# Autodesk Inventor assembly: structure
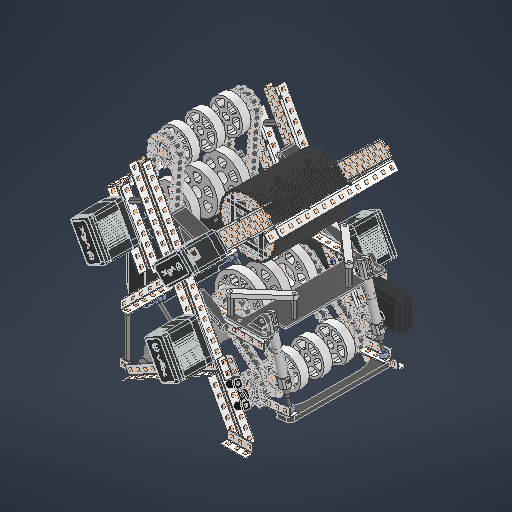
[picture p0: Inventor's stored thumbnail of the model, 512x512]
Saved by Autodesk Inventor 2025.2 (Build 292293000, 293)
## iProperties
Created: 2025-12-03
Part Number: structure
Document SubType Name: Assembly
Designer: cloudy
Mass: 4703.07 g
Surface Area: 21659.1 cm^2
Volume: 2960.96 cm^3
Density: 1.58836 g/cm^3
Author: cloudy
## Documents named in this file (47)
- C:\Users\cloudy\Documents\GitHub\aura-cad\15\structure.iam
- C:\Users\cloudy\Documents\GitHub\aura-cad\!lib\Structure\C Channel\Aluminum 1x3x1 Half\Alu C Half 1x3x1x3.ipt
- C:\Users\cloudy\Documents\GitHub\aura-cad\!lib\Structure\C Channel\Aluminum 1x2x1\Alu C 1x2x1x26.ipt
- C:\Users\cloudy\Documents\GitHub\aura-cad\!lib\Structure\C Channel\Aluminum 1x3x1 Half\Alu C Half 1x3x1x2.ipt
- C:\Users\cloudy\Documents\GitHub\aura-cad\!lib\Structure\C Channel\Aluminum 1x3x1 Half\Alu C Half 1x3x1x12.ipt
- C:\Users\cloudy\Documents\GitHub\aura-cad\!lib\Electronics\Motors with Screws.iam
- C:\Users\cloudy\Documents\GitHub\aura-cad\!lib\Electronics\Motors with Screws\AluM-StarS.iam
- C:\Users\cloudy\Documents\GitHub\aura-cad\!lib\Structure\C Channel\Aluminum 1x2x1\Alu C 1x2x1x14.ipt
- C:\Users\cloudy\Documents\GitHub\aura-cad\15\angleblock.ipt
- C:\Users\cloudy\Documents\GitHub\aura-cad\!lib\Motion\Shaft LS\LS Pillow Bearing Block.ipt
- C:\Users\cloudy\Documents\GitHub\aura-cad\!lib\Structure\C Channel\Aluminum 1x3x1 Half\Alu C Half 1x3x1x17.ipt
- C:\Users\cloudy\Documents\GitHub\aura-cad\!lib\Structure\Standoff\Standoff 1.00.ipt
- C:\Users\cloudy\Documents\GitHub\aura-cad\!lib\Structure\Standoff.ipt
- C:\Users\cloudy\Documents\GitHub\aura-cad\!lib\Structure\C Channel\Aluminum 1x3x1 Half\Alu C Half 1x3x1x8.ipt
- C:\Users\cloudy\Documents\GitHub\aura-cad\15\middlebrace.ipt
- C:\Users\cloudy\Documents\GitHub\aura-cad\15\angleblock_MIR.ipt
- C:\Users\cloudy\Documents\GitHub\aura-cad\15\middlebrace_MIR.ipt
- C:\Users\cloudy\Documents\GitHub\aura-cad\15\ramp.ipt
- C:\Users\cloudy\Documents\GitHub\aura-cad\!lib\Structure\C Channel\Aluminum 1x2x1\Alu C 1x2x1x8.ipt
- C:\Users\cloudy\Documents\GitHub\aura-cad\!lib\Motion\Spacers\Spacer Nylon .375 OD\NSpacer .375 OD x .500.ipt
- C:\Users\cloudy\Documents\GitHub\aura-cad\!lib\Motion\Spacers\Spacer Nylon .375 OD.ipt
- C:\Users\cloudy\Documents\GitHub\aura-cad\!lib\Motion\Spacers\Spacer Nylon .375 OD\NSpacer .375 OD x .125.ipt
- C:\Users\cloudy\Documents\GitHub\aura-cad\!lib\Electronics\V5 Simple Brain.ipt
- C:\Users\cloudy\Documents\GitHub\aura-cad\!lib\Motion\Pneumatics\Legacy - SMC Pneumatics\Reservoir.ipt
- C:\Users\cloudy\Documents\GitHub\aura-cad\!lib\Electronics\V5 Simple Battery.ipt
- C:\Users\cloudy\Documents\GitHub\aura-cad\15\3.157 roller.iam
- C:\Users\cloudy\Documents\GitHub\aura-cad\15\midroller.iam
- C:\Users\cloudy\Documents\GitHub\aura-cad\!lib\Motion\Shaft LS\Shaft Collar Metal\Shaft Collar No Screw.iam
- C:\Users\cloudy\Documents\GitHub\aura-cad\!lib\Motion\Shaft LS\Shaft Collar Metal.iam
- C:\Users\cloudy\Documents\GitHub\aura-cad\15\30 stroke 10 bore\CJ2D10-30Z(0_0).iam
- C:\Users\cloudy\Documents\GitHub\aura-cad\!lib\Structure\Hardware\Nut Keps.ipt
- C:\Users\cloudy\Documents\GitHub\aura-cad\!lib\Motion\Spacers\Spacer Nylon .375 OD\NSpacer .375 OD x .375.ipt
- C:\Users\cloudy\Documents\GitHub\aura-cad\!lib\Motion\Spacers\Washer Steel\SWasher .375 OD x .031250.ipt
- C:\Users\cloudy\Documents\GitHub\aura-cad\!lib\Motion\Spacers\Washer Steel.ipt
- C:\Users\cloudy\Documents\GitHub\aura-cad\!lib\Motion\Shaft LS\Bearing Flat.ipt
- C:\Users\cloudy\Documents\GitHub\aura-cad\!lib\Structure\Hardware\Nut Nylock.ipt
- C:\Users\cloudy\Documents\GitHub\aura-cad\15\back lower roller.iam
- C:\Users\cloudy\Documents\GitHub\aura-cad\15\intake second stage.iam
- C:\Users\cloudy\Documents\GitHub\aura-cad\15\top roller.iam
- C:\Users\cloudy\Documents\GitHub\aura-cad\15\chain 3.256.iam
- C:\Users\cloudy\Documents\GitHub\aura-cad\15\chain 3.48.iam
- C:\Users\cloudy\Documents\GitHub\aura-cad\15\thingy.ipt
- C:\Users\cloudy\Documents\GitHub\aura-cad\!lib\Structure\Standoff\Standoff 2.00.ipt
- C:\Users\cloudy\Documents\GitHub\aura-cad\!lib\Structure\Standoff\Standoff 2.50.ipt
- C:\Users\cloudy\Documents\GitHub\aura-cad\!lib\Structure\C Channel\Aluminum 1x3x1 Half\Alu C Half 1x3x1x6.ipt
- C:\Users\cloudy\Documents\GitHub\aura-cad\15\parkbar.ipt
- C:\Users\cloudy\Documents\GitHub\aura-cad\!lib\Miscellaneous\iw_metal_02.bmp
## Components (91 placed, 40 different names)
1. Alu C Half 1x3x1x3:1 — Insert:2
2. Alu C 1x2x1x26:1 — Insert:2, Insert:4, Insert:6, Mate:3, Insert:7, Mate:4, Insert:9, Insert:11, Mate:5, Insert:12, Mate:6, Insert:15, Insert:18, Insert:19, Insert:43, Insert:49, Insert:50, Insert:51, Insert:52, Insert:77, Insert:114, Insert:115
3. Alu C Half 1x3x1x3:3 — Insert:5, Insert:139
4. Alu C Half 1x3x1x12:1 — Insert:4, Insert:5, Mate:40
5. AluM-StarS:1 [sub-assembly] — Insert:6, Mate:3
6. Alu C 1x2x1x8:2 — Insert:7, Mate:4, Insert:48, Insert:59, Mate:23, Insert:91
7. angleblock:1 — Insert:9, Mate:16
8. Alu C Half 1x3x1x2:2 — Insert:11, Mate:5
9. LS Pillow Bearing Block:1 — Insert:12, Mate:6, Insert:92
10. Alu C Half 1x3x1x6:1 — Insert:15, Insert:71, Insert:82, Mate:29, Insert:88, Mate:136, Flush:1, Insert:143, Mate:137
11. Standoff 1.00:1 — Insert:19
12. Standoff 1.00:2 — Insert:18
13. Alu C Half 1x3x1x3:2 — Insert:22
14. Alu C 1x2x1x26:2 — Insert:22, Insert:24, Mate:8, Insert:25, Mate:9, Insert:26, Insert:29, Mate:11, Insert:30, Mate:12, Insert:31, Insert:37, Insert:38, Insert:44, Insert:53, Insert:54, Insert:55, Insert:56, Insert:64, Insert:78, Insert:93
15. Alu C Half 1x3x1x3:4 — Insert:23, Insert:140
16. Alu C Half 1x3x1x12:3 — Insert:23, Insert:24
17. AluM-StarS:2 [sub-assembly] — Mate:8, Insert:25
18. Alu C 1x2x1x8:1 — Mate:9, Insert:26, Mate:20
19. angleblock_MIR:1 — Insert:29, Mate:17
20. Alu C Half 1x3x1x2:4 — Mate:11, Insert:30
21. LS Pillow Bearing Block:3 — Mate:12, Insert:31
22. Standoff 1.00:3 — Insert:37
23. Standoff 1.00:4 — Insert:38
24. Alu C 1x2x1x14:3 — Insert:45, Mate:18
25. Alu C 1x2x1x14:6 — Insert:43, Mate:16, Mate:18, Insert:58, Mate:22, Insert:61
26. Alu C 1x2x1x14:7 — Insert:44, Mate:17, Insert:45
27. Alu C Half 1x3x1x17:3 — Insert:48, Mate:20
28. NSpacer .375 OD x .500:1 — Insert:49
29. NSpacer .375 OD x .500:2 — Insert:50
30. NSpacer .375 OD x .125:3 — Insert:51
31. NSpacer .375 OD x .125:4 — Insert:52
32. NSpacer .375 OD x .125:5 — Insert:53
33. NSpacer .375 OD x .125:6 — Insert:54
34. NSpacer .375 OD x .500:7 — Insert:55
35. NSpacer .375 OD x .500:8 — Insert:56
36. AluM-StarS:4 [sub-assembly] — Insert:58, Mate:22
37. AluM-StarS:5 [sub-assembly] — Insert:59, Mate:23
38. V5 Simple Brain:1 — Insert:134, Insert:135
39. Reservoir:2 — Tangent:1
40. V5 Simple Battery:1
41. 3.157 roller:2 [sub-assembly] — Insert:61
42. midroller:1 [sub-assembly] — Insert:64, Insert:96, Insert:97
43. Shaft Collar No Screw:1 [sub-assembly] — Insert:71, Insert:117
44. Shaft Collar No Screw:2 [sub-assembly] — Insert:119, Insert:141
45. Nut Keps:1 — Insert:77
46. Nut Keps:2 — Insert:78, Insert:86
47. NSpacer .375 OD x .375:9 — Insert:79, Insert:82
48. SWasher .375 OD x .031250:1 — Insert:79, Insert:80
49. SWasher .375 OD x .031250:2 — Insert:80, Insert:81
50. SWasher .375 OD x .031250:3 — Insert:81
51. NSpacer .375 OD x .375:10 — Mate:135
52. SWasher .375 OD x .031250:4
53. SWasher .375 OD x .031250:5
54. SWasher .375 OD x .031250:6 — Insert:86
55. Bearing Flat:1 — Insert:90, Insert:142, Mate:134
56. Bearing Flat:2 — Mate:29, Insert:88, Insert:89
57. Nut Nylock:1 — Insert:89
58. Nut Nylock:2 — Insert:90, Mate:135
59. back lower roller:1 [sub-assembly] — Insert:91, Mate:30, Insert:95
60. intake second stage:1 [sub-assembly] — Insert:92, Mate:32, Mate:33
61. top roller:1 [sub-assembly] — Insert:93, Insert:94, Mate:31
62. chain 3.256:1 [sub-assembly] — Insert:94, Mate:30
63. chain 3.256:2 [sub-assembly] — Insert:95, Mate:31
64. chain 3.48:1 [sub-assembly] — Insert:96, Mate:32
65. chain 3.48:2 [sub-assembly] — Mate:33, Insert:97
66. middlebrace:2 — Insert:115, Mate:38
67. Alu C Half 1x3x1x8:3 — Insert:114
68. middlebrace_MIR:2 — Mate:38
69. Alu C Half 1x3x1x8:4 — Insert:120
70. ramp:2 — Insert:116, Insert:118, Insert:120, Insert:121, Insert:122, Insert:123, Insert:124
71. thingy:3
72. thingy:4
73. CJ2D10-30Z(0_0):1 [sub-assembly] — Insert:116, Insert:117
74. CJ2D10-30Z(0_0):2 [sub-assembly] — Insert:118, Insert:119
75. Standoff 1.00:6 — Insert:123
76. Standoff 1.00:7 — Insert:122
77. Standoff 1.00:8 — Insert:124
78. Standoff 1.00:9 — Insert:121
79. Shaft Collar No Screw:3 [sub-assembly] — Insert:127, Insert:128
80. Shaft Collar No Screw:4 [sub-assembly] — Insert:127, Insert:133
81. Standoff 2.00:10 — Insert:128, Mate:130
82. Shaft Collar No Screw:5 [sub-assembly] — Mate:130, Mate:40, Mate:41, Tangent:1
83. Shaft Collar No Screw:6 [sub-assembly]
84. Shaft Collar No Screw:7 [sub-assembly] — Insert:136
85. Standoff 2.00:11 — Mate:133
86. Shaft Collar No Screw:8 [sub-assembly] — Mate:133, Mate:41
87. Alu C Half 1x3x1x17:4 — Insert:133, Insert:134, Insert:135, Insert:136, Insert:137, Insert:138
88. Standoff 2.50:12 — Insert:137, Insert:140
89. Standoff 2.50:13 — Insert:138, Insert:139
90. Alu C Half 1x3x1x6:2 — Insert:141, Insert:142, Mate:134, Mate:136
91. parkbar:1 — Flush:1, Insert:143, Mate:137
## Relationships (122: Insert 90, Mate 30, Tangent 1, Flush 1)
- Insert:2 (12.7 mm): Alu C Half 1x3x1x3:1 ↔ Alu C 1x2x1x26:1
- Insert:4 (12.7 mm): Alu C 1x2x1x26:1 ↔ Alu C Half 1x3x1x12:1
- Insert:5: Alu C Half 1x3x1x3:3 ↔ Alu C Half 1x3x1x12:1
- Insert:6: Alu C 1x2x1x26:1 ↔ AluM-StarS:1
- Mate:3: Alu C 1x2x1x26:1 ↔ AluM-StarS:1
- Insert:7 (25.4 mm): Alu C 1x2x1x26:1 ↔ Alu C 1x2x1x8:2
- Mate:4: Alu C 1x2x1x26:1 ↔ Alu C 1x2x1x8:2
- Insert:9: Alu C 1x2x1x26:1 ↔ angleblock:1
- Insert:11 (3.175 mm): Alu C 1x2x1x26:1 ↔ Alu C Half 1x3x1x2:2
- Mate:5: Alu C 1x2x1x26:1 ↔ Alu C Half 1x3x1x2:2
- Insert:12 (12.7 mm): Alu C 1x2x1x26:1 ↔ LS Pillow Bearing Block:1
- Mate:6: Alu C 1x2x1x26:1 ↔ LS Pillow Bearing Block:1
- Insert:15 (15.875 mm): Alu C 1x2x1x26:1 ↔ Alu C Half 1x3x1x6:1
- Insert:18: Alu C 1x2x1x26:1 ↔ Standoff 1.00:2
- Insert:19: Alu C 1x2x1x26:1 ↔ Standoff 1.00:1
- Insert:22 (12.7 mm): Alu C Half 1x3x1x3:2 ↔ Alu C 1x2x1x26:2
- Insert:23: Alu C Half 1x3x1x3:4 ↔ Alu C Half 1x3x1x12:3
- Insert:24 (12.7 mm): Alu C 1x2x1x26:2 ↔ Alu C Half 1x3x1x12:3
- Mate:8: Alu C 1x2x1x26:2 ↔ AluM-StarS:2
- Insert:25: Alu C 1x2x1x26:2 ↔ AluM-StarS:2
- Mate:9: Alu C 1x2x1x26:2 ↔ Alu C 1x2x1x8:1
- Insert:26 (25.4 mm): Alu C 1x2x1x26:2 ↔ Alu C 1x2x1x8:1
- Insert:29: Alu C 1x2x1x26:2 ↔ angleblock_MIR:1
- Mate:11: Alu C 1x2x1x26:2 ↔ Alu C Half 1x3x1x2:4
- Insert:30 (3.175 mm): Alu C 1x2x1x26:2 ↔ Alu C Half 1x3x1x2:4
- Mate:12: Alu C 1x2x1x26:2 ↔ LS Pillow Bearing Block:3
- Insert:31 (12.7 mm): Alu C 1x2x1x26:2 ↔ LS Pillow Bearing Block:3
- Insert:37: Alu C 1x2x1x26:2 ↔ Standoff 1.00:3
- Insert:38: Alu C 1x2x1x26:2 ↔ Standoff 1.00:4
- Insert:43 (3.175 mm): Alu C 1x2x1x26:1 ↔ Alu C 1x2x1x14:6
- Mate:16: angleblock:1 ↔ Alu C 1x2x1x14:6
- Insert:44 (3.175 mm): Alu C 1x2x1x26:2 ↔ Alu C 1x2x1x14:7
- Mate:17: angleblock_MIR:1 ↔ Alu C 1x2x1x14:7
- Insert:45: Alu C 1x2x1x14:3 ↔ Alu C 1x2x1x14:7
- Mate:18: Alu C 1x2x1x14:3 ↔ Alu C 1x2x1x14:6
- Insert:48: Alu C 1x2x1x8:2 ↔ Alu C Half 1x3x1x17:3
- Mate:20: Alu C 1x2x1x8:1 ↔ Alu C Half 1x3x1x17:3
- Insert:49: Alu C 1x2x1x26:1 ↔ NSpacer .375 OD x .500:1
- Insert:50: Alu C 1x2x1x26:1 ↔ NSpacer .375 OD x .500:2
- Insert:51: Alu C 1x2x1x26:1 ↔ NSpacer .375 OD x .125:3
- Insert:52: Alu C 1x2x1x26:1 ↔ NSpacer .375 OD x .125:4
- Insert:53: Alu C 1x2x1x26:2 ↔ NSpacer .375 OD x .125:5
- Insert:54: Alu C 1x2x1x26:2 ↔ NSpacer .375 OD x .125:6
- Insert:55: Alu C 1x2x1x26:2 ↔ NSpacer .375 OD x .500:7
- Insert:56: Alu C 1x2x1x26:2 ↔ NSpacer .375 OD x .500:8
- Insert:58: Alu C 1x2x1x14:6 ↔ AluM-StarS:4
- Mate:22: Alu C 1x2x1x14:6 ↔ AluM-StarS:4
- Insert:59: Alu C 1x2x1x8:2 ↔ AluM-StarS:5
- Mate:23: Alu C 1x2x1x8:2 ↔ AluM-StarS:5
- Insert:61 (29.1465 mm): Alu C 1x2x1x14:6 ↔ 3.157 roller:2
- Insert:64 (32.7025 mm): Alu C 1x2x1x26:2 ↔ midroller:1
- Insert:71: Alu C Half 1x3x1x6:1 ↔ Shaft Collar No Screw:1
- Insert:77: Alu C 1x2x1x26:1 ↔ Nut Keps:1
- Insert:78: Alu C 1x2x1x26:2 ↔ Nut Keps:2
- Insert:79: NSpacer .375 OD x .375:9 ↔ SWasher .375 OD x .031250:1
- Insert:80: SWasher .375 OD x .031250:1 ↔ SWasher .375 OD x .031250:2
- Insert:81: SWasher .375 OD x .031250:2 ↔ SWasher .375 OD x .031250:3
- Insert:82: Alu C Half 1x3x1x6:1 ↔ NSpacer .375 OD x .375:9
- [Insert]: NSpacer .375 OD x .375:10 ↔ SWasher .375 OD x .031250:4
- [Insert]: SWasher .375 OD x .031250:4 ↔ SWasher .375 OD x .031250:5
- [Insert]: SWasher .375 OD x .031250:5 ↔ SWasher .375 OD x .031250:6
- Insert:86: Nut Keps:2 ↔ SWasher .375 OD x .031250:6
- Mate:29: Alu C Half 1x3x1x6:1 ↔ Bearing Flat:2
- Insert:88: Alu C Half 1x3x1x6:1 ↔ Bearing Flat:2
- Insert:89: Bearing Flat:2 ↔ Nut Nylock:1
- Insert:90: Bearing Flat:1 ↔ Nut Nylock:2
- Insert:91 (29.5275 mm): Alu C 1x2x1x8:2 ↔ back lower roller:1
- Insert:92 (5.08 mm): LS Pillow Bearing Block:1 ↔ intake second stage:1
- Insert:93 (29.5275 mm): Alu C 1x2x1x26:2 ↔ top roller:1
- Insert:94: top roller:1 ↔ chain 3.256:1
- Mate:30: back lower roller:1 ↔ chain 3.256:1
- Insert:95: back lower roller:1 ↔ chain 3.256:2
- Mate:31: top roller:1 ↔ chain 3.256:2
- Insert:96: midroller:1 ↔ chain 3.48:1
- Mate:32: intake second stage:1 ↔ chain 3.48:1
- Mate:33: intake second stage:1 ↔ chain 3.48:2
- Insert:97: midroller:1 ↔ chain 3.48:2
- [Insert]: middlebrace_MIR:2 ↔ Alu C Half 1x3x1x8:4
- [Insert]: middlebrace:2 ↔ Alu C Half 1x3x1x8:3
- [Insert]: Alu C Half 1x3x1x8:3 ↔ ramp:2
- [Insert]: Alu C Half 1x3x1x8:3 ↔ ramp:2
- [Mate]: Alu C Half 1x3x1x8:4 ↔ ramp:2
- [Insert] (25.4 mm): ramp:2 ↔ thingy:3
- [Insert] (25.4 mm): ramp:2 ↔ thingy:4
- [Mate]: ramp:2 ↔ thingy:4
- Insert:114: Alu C 1x2x1x26:1 ↔ Alu C Half 1x3x1x8:3
- Insert:115: Alu C 1x2x1x26:1 ↔ middlebrace:2
- Mate:38: middlebrace:2 ↔ middlebrace_MIR:2
- Insert:116: ramp:2 ↔ CJ2D10-30Z(0_0):1
- Insert:117: Shaft Collar No Screw:1 ↔ CJ2D10-30Z(0_0):1
- Insert:118: ramp:2 ↔ CJ2D10-30Z(0_0):2
- Insert:119: Shaft Collar No Screw:2 ↔ CJ2D10-30Z(0_0):2
- Insert:120: Alu C Half 1x3x1x8:4 ↔ ramp:2
- Insert:121: ramp:2 ↔ Standoff 1.00:9
- Insert:122: ramp:2 ↔ Standoff 1.00:7
- Insert:123: ramp:2 ↔ Standoff 1.00:6
- Insert:124: ramp:2 ↔ Standoff 1.00:8
- Insert:127: Shaft Collar No Screw:3 ↔ Shaft Collar No Screw:4
- Insert:128: Shaft Collar No Screw:3 ↔ Standoff 2.00:10
- Mate:130: Standoff 2.00:10 ↔ Shaft Collar No Screw:5
- Mate:40: Alu C Half 1x3x1x12:1 ↔ Shaft Collar No Screw:5
- [Insert]: Shaft Collar No Screw:6 ↔ Shaft Collar No Screw:7
- [Insert]: Shaft Collar No Screw:6 ↔ Standoff 2.00:11
- Mate:133: Standoff 2.00:11 ↔ Shaft Collar No Screw:8
- Mate:41: Shaft Collar No Screw:5 ↔ Shaft Collar No Screw:8
- Insert:133: Shaft Collar No Screw:4 ↔ Alu C Half 1x3x1x17:4
- Insert:134: V5 Simple Brain:1 ↔ Alu C Half 1x3x1x17:4
- Insert:135: V5 Simple Brain:1 ↔ Alu C Half 1x3x1x17:4
- Insert:136: Shaft Collar No Screw:7 ↔ Alu C Half 1x3x1x17:4
- Tangent:1: Reservoir:2 ↔ Shaft Collar No Screw:5
- Insert:137: Alu C Half 1x3x1x17:4 ↔ Standoff 2.50:12
- Insert:138: Alu C Half 1x3x1x17:4 ↔ Standoff 2.50:13
- Insert:139 (9.525 mm): Alu C Half 1x3x1x3:3 ↔ Standoff 2.50:13
- Insert:140 (9.525 mm): Alu C Half 1x3x1x3:4 ↔ Standoff 2.50:12
- Insert:141: Shaft Collar No Screw:2 ↔ Alu C Half 1x3x1x6:2
- Insert:142: Bearing Flat:1 ↔ Alu C Half 1x3x1x6:2
- Mate:134: Bearing Flat:1 ↔ Alu C Half 1x3x1x6:2
- Mate:135: NSpacer .375 OD x .375:10 ↔ Nut Nylock:2
- Mate:136: Alu C Half 1x3x1x6:1 ↔ Alu C Half 1x3x1x6:2
- Flush:1: Alu C Half 1x3x1x6:1 ↔ parkbar:1
- Insert:143: Alu C Half 1x3x1x6:1 ↔ parkbar:1
- Mate:137: Alu C Half 1x3x1x6:1 ↔ parkbar:1
## Named parameters: d145_d141 = 0 mm, d146_d142 = 0 mm, d147_d143 = 0 mm, d183_d174 = 0 mm, d184_d175 = 0 mm, d185_d176 = 0 mm, d186_d177 = 0 mm, d187_d178 = 0 mm, d188_d180 = 25.4 mm, d189_d181 = 25.4 mm, d190_d182 = 0 mm, d210_d206 = 0 mm, d211_d207 = 0 mm, d212_d208 = 0 mm
